# Autodesk Inventor assembly: Assy_cover_front
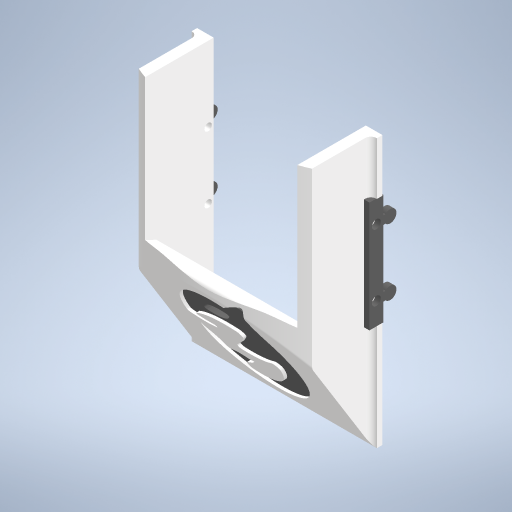
[picture p0: Inventor's stored thumbnail of the model, 512x512]
Saved by Autodesk Inventor 2024.1 (Build 281209000, 209)
## iProperties
Created: 2025-03-07
Part Number: Assy_cover_front
Document SubType Name: Assembly
Designer: hibik
Author: hibik
## Documents named in this file (4)
- C:\Users\hibik\Documents\Robomech\RESCUE\ORCA\hard\cover\Assy_cover_front.iam
- C:\Users\hibik\Documents\Robomech\RESCUE\ORCA\hard\cover\cover_front.ipt
- C:\Users\hibik\Documents\Robomech\RESCUE\ORCA\hard\cover\cover_setter.ipt
- C:\Users\hibik\Documents\Robomech\RESCUE\ORCA\hard\cover\ROGO_front_cover.ipt
## Components (4 placed, 3 different names)
1. cover_front:1 — フラッシュ:3, 挿入:1, 挿入:2, 挿入:3, 挿入:4
2. ROGO_front_cover:1 — フラッシュ:2, フラッシュ:3
3. cover_setter:2 — 挿入:1, 挿入:2
4. cover_setter:3 — 挿入:3, 挿入:4
## Relationships (6: Insert 4, Flush 2)
- フラッシュ:2 [Flush]: ROGO_front_cover:1
- フラッシュ:3 [Flush] (23 mm): cover_front:1 ↔ ROGO_front_cover:1
- 挿入:1 [Insert]: cover_front:1 ↔ cover_setter:2
- 挿入:2 [Insert]: cover_front:1 ↔ cover_setter:2
- 挿入:3 [Insert]: cover_front:1 ↔ cover_setter:3
- 挿入:4 [Insert]: cover_front:1 ↔ cover_setter:3
